# Autodesk Inventor assembly: Assembly_Opentrons_Imagingunit_v1
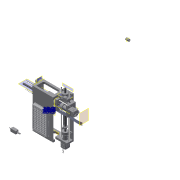
[picture p0: Inventor's stored thumbnail of the model, 180x180]
Saved by Autodesk Inventor 2019.4 (Build 234330000, 330)
## iProperties
Created: 2020-10-27
Part Number: Assembly_Opentrons_Imagingunit_v1
Document SubType Name: Assembly
Designer: diederichbenedict
Author: diederichbenedict
## Documents named in this file (13)
- C:\Users\diederichbenedict\Dropbox\Dokumente\Promotion\PROJECTS\OPENTRONS\INVENTOR\Assembly_Opentrons_Imagingunit_v1.iam
- C:\Users\diederichbenedict\Dropbox\Dokumente\Promotion\PROJECTS\OPENTRONS\INVENTOR\Assembly_Opentrons_Autofocus_v0.iam
- C:\Users\diederichbenedict\Dropbox\Dokumente\Promotion\PROJECTS\OPENTRONS\INVENTOR\00_MTP_96-welplate.ipt
- C:\Users\diederichbenedict\Dropbox\Dokumente\Promotion\PROJECTS\OPENTRONS\INVENTOR\00_IGUS_Drylin_RJ4JP-01-06.ipt
- C:\Users\diederichbenedict\Dropbox\Dokumente\Promotion\PROJECTS\OPENTRONS\INVENTOR\04_OPENTRONS_Microscope_wellplate_base.ipt
- C:\Users\diederichbenedict\Dropbox\Dokumente\Promotion\PROJECTS\OPENTRONS\INVENTOR\Assembly_opentrons_microscope_slide_y.iam
- C:\Users\diederichbenedict\Dropbox\Dokumente\Promotion\PROJECTS\OPENTRONS\INVENTOR\Assembly_opentrons_microscope_slide_y_base.iam
- C:\Users\diederichbenedict\Dropbox\Dokumente\Promotion\PROJECTS\OPENTRONS\INVENTOR\00_Endstop.ipt
- C:\Users\diederichbenedict\Dropbox\Dokumente\Promotion\PROJECTS\OPENTRONS\INVENTOR\00_3rdleg.ipt
- C:\Users\diederichbenedict\Dropbox\Dokumente\Promotion\PROJECTS\OPENTRONS\INVENTOR\06_OPENTRONS_Microscope_Extraslide.ipt
- C:\Users\diederichbenedict\Dropbox\Dokumente\Promotion\PROJECTS\OPENTRONS\INVENTOR\00_Thorlabs_Rod_200mm.ipt
- C:\Users\diederichbenedict\Dropbox\Dokumente\Promotion\PROJECTS\OPENTRONS\INVENTOR\06_OPENTRONS_Microscope_Extraslide_slide.ipt
- C:\Users\diederichbenedict\Dropbox\Dokumente\Promotion\PROJECTS\OPENTRONS\INVENTOR\00_JF-0530B-solenoid.ipt
## Components (12 placed, 12 different names)
1. 00_IGUS_Drylin_RJ4JP-01-06:9
2. 04_OPENTRONS_Microscope_wellplate_base:1 — Mate:8, Mate:9, Mate:10, Insert:1
3. Assembly_Opentrons_Autofocus_v0:1 [sub-assembly] — Mate:3, Mate:4
4. Assembly_opentrons_microscope_slide_y:1 [sub-assembly] — Mate:1, Mate:2, Mate:3, Mate:4, Mate:12
5. Assembly_opentrons_microscope_slide_y_base:1 [sub-assembly] — Mate:1, Flush:7, Flush:8, Flush:9, Mate:2, Mate:6, Mate:7, Mate:11, Insert:1, Angle:1, Flush:10, Flush:11, Flush:12, Flush:13, Flush:14
6. 00_MTP_96-welplate:1 — Mate:6, Mate:7, Mate:8, Mate:9, Mate:10
7. 00_Endstop:1 — Mate:11, Mate:12, Angle:1, Flush:10
8. 00_3rdleg:1 — Flush:11, Flush:12
9. 06_OPENTRONS_Microscope_Extraslide:1 — Flush:13, Flush:14, Insert:2, Flush:15, Flush:16
10. 00_Thorlabs_Rod_200mm:1 — Insert:2
11. 06_OPENTRONS_Microscope_Extraslide_slide:1 — Flush:15, Flush:16
12. 00_JF-0530B-solenoid:1
## Relationships (24: Mate 11, Flush 10, Insert 2, Angle 1)
- Mate:1: Assembly_opentrons_microscope_slide_y:1 ↔ Assembly_opentrons_microscope_slide_y_base:1
- Flush:7: Assembly_opentrons_microscope_slide_y_base:1
- Flush:8: Assembly_opentrons_microscope_slide_y_base:1
- Flush:9: Assembly_opentrons_microscope_slide_y_base:1
- Mate:2: Assembly_opentrons_microscope_slide_y:1 ↔ Assembly_opentrons_microscope_slide_y_base:1
- Mate:3: Assembly_Opentrons_Autofocus_v0:1 ↔ Assembly_opentrons_microscope_slide_y:1
- Mate:4: Assembly_Opentrons_Autofocus_v0:1 ↔ Assembly_opentrons_microscope_slide_y:1
- Mate:6 (8 mm): Assembly_opentrons_microscope_slide_y_base:1 ↔ 00_MTP_96-welplate:1
- Mate:7 (18 mm): Assembly_opentrons_microscope_slide_y_base:1 ↔ 00_MTP_96-welplate:1
- Mate:8: 04_OPENTRONS_Microscope_wellplate_base:1 ↔ 00_MTP_96-welplate:1
- Mate:9 (-2 mm): 04_OPENTRONS_Microscope_wellplate_base:1 ↔ 00_MTP_96-welplate:1
- Mate:10 (-2 mm): 04_OPENTRONS_Microscope_wellplate_base:1 ↔ 00_MTP_96-welplate:1
- Mate:11: Assembly_opentrons_microscope_slide_y_base:1 ↔ 00_Endstop:1
- Insert:1: 04_OPENTRONS_Microscope_wellplate_base:1 ↔ Assembly_opentrons_microscope_slide_y_base:1
- Mate:12: Assembly_opentrons_microscope_slide_y:1 ↔ 00_Endstop:1
- Angle:1 (180 deg): Assembly_opentrons_microscope_slide_y_base:1 ↔ 00_Endstop:1
- Flush:10 (10 mm): Assembly_opentrons_microscope_slide_y_base:1 ↔ 00_Endstop:1
- Flush:11: Assembly_opentrons_microscope_slide_y_base:1 ↔ 00_3rdleg:1
- Flush:12: Assembly_opentrons_microscope_slide_y_base:1 ↔ 00_3rdleg:1
- Flush:13: Assembly_opentrons_microscope_slide_y_base:1 ↔ 06_OPENTRONS_Microscope_Extraslide:1
- Flush:14: Assembly_opentrons_microscope_slide_y_base:1 ↔ 06_OPENTRONS_Microscope_Extraslide:1
- Insert:2: 06_OPENTRONS_Microscope_Extraslide:1 ↔ 00_Thorlabs_Rod_200mm:1
- Flush:15: 06_OPENTRONS_Microscope_Extraslide:1 ↔ 06_OPENTRONS_Microscope_Extraslide_slide:1
- Flush:16: 06_OPENTRONS_Microscope_Extraslide:1 ↔ 06_OPENTRONS_Microscope_Extraslide_slide:1
